# Autodesk Inventor assembly: Flywheel Assembly
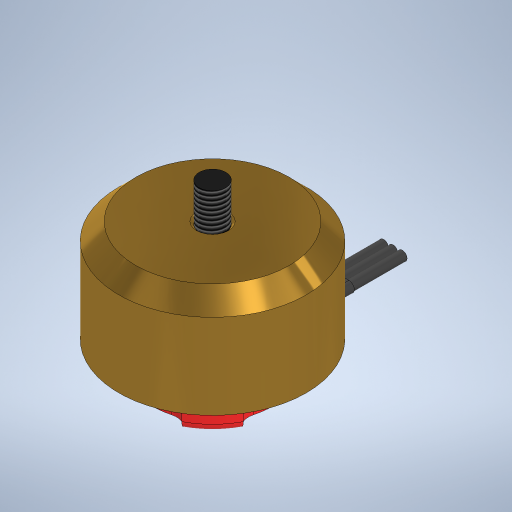
[picture p0: Inventor's stored thumbnail of the model, 512x512]
Saved by Autodesk Inventor 2023.4 (Build 274418000, 418)
## iProperties
Created: 2024-05-27
Part Number: Flywheel Assembly
Document SubType Name: Assembly
Designer: Nathan Cai
Mass: 28.8 g
Surface Area: 159.199 cm^2
Volume: 16.2986 cm^3
Density: 1.76703 g/cm^3
Author: Nathan Cai
## Documents named in this file (3)
- E:\Documents\Inventor\Chort V2.1\Flywheel Assembly.iam
- E:\Documents\Inventor\Chort V2.1\AKK RS2205 2300KV\AKK RS2205 2300KV.iam
- E:\Documents\Inventor\Chort V2.1\Flywheel.ipt
## Components (2 placed, 2 different names)
1. AKK RS2205 2300KV:1 [sub-assembly] — Mate:1, Mate:2
2. Flywheel:1 — Mate:1, Mate:2
## Relationships (2: Mate 2)
- Mate:1: AKK RS2205 2300KV:1 ↔ Flywheel:1
- Mate:2: AKK RS2205 2300KV:1 ↔ Flywheel:1
